# Autodesk Inventor assembly: CL7-GB-100
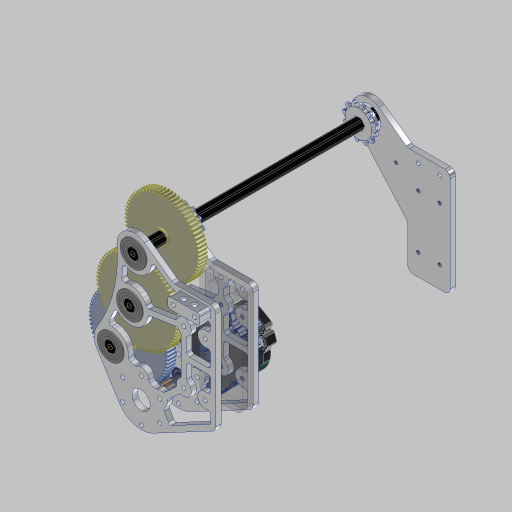
[picture p0: Inventor's stored thumbnail of the model, 512x512]
Saved by Autodesk Inventor 2023.5 (Build 275446000, 446)
## iProperties
Created: 2025-03-18
Part Number: CL7-GB-100
Document SubType Name: Assembly
Designer: slick
Mass: 1483.84 g
Surface Area: 2349.97 cm^2
Volume: 652.786 cm^3
Density: 2.27309 g/cm^3
Author: slick
## Documents named in this file (17)
- C:\Users\slick\OneDrive\Desktop\2025-ReefScape---CAD\Climber\CL7\CL-GB\CL7-GB-100.iam
- C:\Users\slick\OneDrive\Desktop\2025-ReefScape---CAD\Climber\CL7\CL-GB\CL7-GB-001.ipt
- C:\Users\slick\OneDrive\Desktop\2025-ReefScape---CAD\Climber\CL7\CL-GB\CL7-GB-002.ipt
- C:\Users\slick\OneDrive\Desktop\2025-ReefScape---CAD\Climber\CL7\CL-GB\CL7-GB-003.ipt
- C:\Users\slick\OneDrive\Desktop\2025-ReefScape---CAD\COMMON PARTS\MOTORS\Kracken with Cover and Boards.iam
- C:\Users\slick\OneDrive\Desktop\2025-ReefScape---CAD\COMMON PARTS\BEARINGS\13_75mm_1_2_ThunderHex_ID_x_1_125_OD_x_0_313_WD_Flanged_Bearing_217-4006_MIR.ipt
- C:\Users\slick\OneDrive\Desktop\2025-ReefScape---CAD\COMMON PARTS\GEARS\20dp .5 hex\72t_Aluminum_Spur_Gear_20_DP_1_2_Hex_Bore_217-3576.ipt
- C:\Users\slick\OneDrive\Desktop\2025-ReefScape---CAD\COMMON PARTS\GEARS\20dp .5 hex\18t_Aluminum_Spur_Gear_20_DP_1_2_Hex_Bore_217-3209.ipt
- C:\Users\slick\OneDrive\Desktop\2025-ReefScape---CAD\COMMON PARTS\GEARS\20dp .5 hex\74t_Aluminum_Spur_Gear_20_DP_1_2_Hex_Bore_217-5478.ipt
- C:\Users\slick\OneDrive\Desktop\2025-ReefScape---CAD\COMMON PARTS\GEARS\20dp .5 hex\20t_Aluminum_Spur_Gear_20_DP_1_2_Hex_Bore_217-2702.ipt
- C:\Users\slick\OneDrive\Desktop\2025-ReefScape---CAD\COMMON PARTS\GEARS\20dp .5 hex\68t_Aluminum_Spur_Gear_20_DP_1_2_Hex_Bore_217-5477.ipt
- C:\Users\slick\OneDrive\Desktop\2025-ReefScape---CAD\COMMON PARTS\GEARS\WCP-1006\WCP-1006.ipt
- C:\Users\slick\OneDrive\Desktop\2025-ReefScape---CAD\Climber\CL7\CL-GB\CL7-GB-004.ipt
- C:\Users\slick\OneDrive\Desktop\2025-ReefScape---CAD\COMMON PARTS\SPROCKETS\35\12t_Aluminum_Hub_Sprocket_35_Chain_1_2_Hex_Bore_217-2662.ipt
- C:\Users\slick\OneDrive\Desktop\2025-ReefScape---CAD\Climber\CL7\CL-GB\CL7-GB-006.ipt
- C:\Users\slick\OneDrive\Desktop\2025-ReefScape---CAD\Climber\CL7\CL-GB\CL7-GB-007.ipt
- C:\Users\slick\OneDrive\Desktop\2025-ReefScape---CAD\Climber\CL7\CL-GB\CL7-GB-008.ipt
## Components (24 placed, 16 different names)
1. CL7-GB-001:1 — Mate:2, Insert:6, Insert:7, Insert:8, Flush:5, Mate:18, Mate:19, Insert:14, Insert:15, Insert:16, Mate:23, Flush:12, Mate:34
2. CL7-GB-002:1 — Mate:2, Flush:1, Insert:9, Insert:10, Insert:11, Flush:5, Mate:23, Insert:17, Insert:18, Mate:33
3. CL7-GB-003:1 — Insert:1, Insert:2, Flush:1, Insert:15, Insert:16
4. CL7-GB-003:2 — Insert:1, Insert:2
5. Kracken with Cover and Boards:1 [sub-assembly] — Mate:18, Mate:19, Insert:14, Mate:20
6. 13_75mm_1_2_ThunderHex_ID_x_1_125_OD_x_0_313_WD_Flanged_Bearing_217-4006_MIR:1 — Insert:8, Mate:5, Mate:27, Flush:6
7. 13_75mm_1_2_ThunderHex_ID_x_1_125_OD_x_0_313_WD_Flanged_Bearing_217-4006_MIR:2 — Insert:7, Mate:28, Flush:7
8. 13_75mm_1_2_ThunderHex_ID_x_1_125_OD_x_0_313_WD_Flanged_Bearing_217-4006_MIR:3 — Insert:6, Mate:21, Mate:24
9. 13_75mm_1_2_ThunderHex_ID_x_1_125_OD_x_0_313_WD_Flanged_Bearing_217-4006_MIR:4 — Insert:11, Mate:12, Mate:29, Mate:30, Flush:11
10. 13_75mm_1_2_ThunderHex_ID_x_1_125_OD_x_0_313_WD_Flanged_Bearing_217-4006_MIR:5 — Insert:10, Mate:9, Mate:10, Mate:26
11. 13_75mm_1_2_ThunderHex_ID_x_1_125_OD_x_0_313_WD_Flanged_Bearing_217-4006_MIR:6 — Insert:9
12. 72t_Aluminum_Spur_Gear_20_DP_1_2_Hex_Bore_217-3576:1 — Mate:5, Mate:7, Flush:4, Mate:22
13. 18t_Aluminum_Spur_Gear_20_DP_1_2_Hex_Bore_217-3209:1 — Mate:7, Flush:2, Mate:22
14. 74t_Aluminum_Spur_Gear_20_DP_1_2_Hex_Bore_217-5478:1 — Mate:9, Flush:2, Mate:26
15. 20t_Aluminum_Spur_Gear_20_DP_1_2_Hex_Bore_217-2702:1 — Mate:10, Flush:3
16. 68t_Aluminum_Spur_Gear_20_DP_1_2_Hex_Bore_217-5477:1 — Mate:12, Flush:3, Mate:21
17. WCP-1006:1 — Flush:4, Mate:20
18. CL7-GB-004:1 — Insert:17, Insert:18
19. 12t_Aluminum_Hub_Sprocket_35_Chain_1_2_Hex_Bore_217-2662:1 — Mate:24, Mate:29
20. CL7-GB-006:1 — Mate:27, Flush:6
21. CL7-GB-006:2 — Mate:28, Flush:7
22. CL7-GB-007:1 — Mate:30, Flush:11, Mate:32
23. 12t_Aluminum_Hub_Sprocket_35_Chain_1_2_Hex_Bore_217-2662:2 — Mate:32
24. CL7-GB-008:1 — Mate:33, Flush:12, Mate:34
## Relationships (43: Mate 21, Insert 13, Flush 9)
- Insert:1: CL7-GB-003:1 ↔ CL7-GB-003:2
- Insert:2: CL7-GB-003:1 ↔ CL7-GB-003:2
- Mate:2: CL7-GB-001:1 ↔ CL7-GB-002:1
- Flush:1: CL7-GB-002:1 ↔ CL7-GB-003:1
- Insert:6: CL7-GB-001:1 ↔ 13_75mm_1_2_ThunderHex_ID_x_1_125_OD_x_0_313_WD_Flanged_Bearing_217-4006_MIR:3
- Insert:7: CL7-GB-001:1 ↔ 13_75mm_1_2_ThunderHex_ID_x_1_125_OD_x_0_313_WD_Flanged_Bearing_217-4006_MIR:2
- Insert:8: CL7-GB-001:1 ↔ 13_75mm_1_2_ThunderHex_ID_x_1_125_OD_x_0_313_WD_Flanged_Bearing_217-4006_MIR:1
- Insert:9: CL7-GB-002:1 ↔ 13_75mm_1_2_ThunderHex_ID_x_1_125_OD_x_0_313_WD_Flanged_Bearing_217-4006_MIR:6
- Insert:10: CL7-GB-002:1 ↔ 13_75mm_1_2_ThunderHex_ID_x_1_125_OD_x_0_313_WD_Flanged_Bearing_217-4006_MIR:5
- Insert:11: CL7-GB-002:1 ↔ 13_75mm_1_2_ThunderHex_ID_x_1_125_OD_x_0_313_WD_Flanged_Bearing_217-4006_MIR:4
- Mate:5: 13_75mm_1_2_ThunderHex_ID_x_1_125_OD_x_0_313_WD_Flanged_Bearing_217-4006_MIR:1 ↔ 72t_Aluminum_Spur_Gear_20_DP_1_2_Hex_Bore_217-3576:1
- Mate:7: 72t_Aluminum_Spur_Gear_20_DP_1_2_Hex_Bore_217-3576:1 ↔ 18t_Aluminum_Spur_Gear_20_DP_1_2_Hex_Bore_217-3209:1
- Mate:9: 13_75mm_1_2_ThunderHex_ID_x_1_125_OD_x_0_313_WD_Flanged_Bearing_217-4006_MIR:5 ↔ 74t_Aluminum_Spur_Gear_20_DP_1_2_Hex_Bore_217-5478:1
- Flush:2: 18t_Aluminum_Spur_Gear_20_DP_1_2_Hex_Bore_217-3209:1 ↔ 74t_Aluminum_Spur_Gear_20_DP_1_2_Hex_Bore_217-5478:1
- Mate:10: 13_75mm_1_2_ThunderHex_ID_x_1_125_OD_x_0_313_WD_Flanged_Bearing_217-4006_MIR:5 ↔ 20t_Aluminum_Spur_Gear_20_DP_1_2_Hex_Bore_217-2702:1
- Mate:12: 13_75mm_1_2_ThunderHex_ID_x_1_125_OD_x_0_313_WD_Flanged_Bearing_217-4006_MIR:4 ↔ 68t_Aluminum_Spur_Gear_20_DP_1_2_Hex_Bore_217-5477:1
- Flush:3: 20t_Aluminum_Spur_Gear_20_DP_1_2_Hex_Bore_217-2702:1 ↔ 68t_Aluminum_Spur_Gear_20_DP_1_2_Hex_Bore_217-5477:1
- Flush:4 (6.35 mm): 72t_Aluminum_Spur_Gear_20_DP_1_2_Hex_Bore_217-3576:1 ↔ WCP-1006:1
- Flush:5: CL7-GB-001:1 ↔ CL7-GB-002:1
- Mate:18: CL7-GB-001:1 ↔ Kracken with Cover and Boards:1
- Mate:19: CL7-GB-001:1 ↔ Kracken with Cover and Boards:1
- Insert:14: CL7-GB-001:1 ↔ Kracken with Cover and Boards:1
- Mate:20: Kracken with Cover and Boards:1 ↔ WCP-1006:1
- Mate:21: 13_75mm_1_2_ThunderHex_ID_x_1_125_OD_x_0_313_WD_Flanged_Bearing_217-4006_MIR:3 ↔ 68t_Aluminum_Spur_Gear_20_DP_1_2_Hex_Bore_217-5477:1
- Mate:22: 72t_Aluminum_Spur_Gear_20_DP_1_2_Hex_Bore_217-3576:1 ↔ 18t_Aluminum_Spur_Gear_20_DP_1_2_Hex_Bore_217-3209:1
- Insert:15: CL7-GB-001:1 ↔ CL7-GB-003:1
- Insert:16: CL7-GB-001:1 ↔ CL7-GB-003:1
- Mate:23 (38.1 mm): CL7-GB-001:1 ↔ CL7-GB-002:1
- Insert:17: CL7-GB-002:1 ↔ CL7-GB-004:1
- Insert:18: CL7-GB-002:1 ↔ CL7-GB-004:1
- Mate:24: 13_75mm_1_2_ThunderHex_ID_x_1_125_OD_x_0_313_WD_Flanged_Bearing_217-4006_MIR:3 ↔ 12t_Aluminum_Hub_Sprocket_35_Chain_1_2_Hex_Bore_217-2662:1
- Mate:26: 13_75mm_1_2_ThunderHex_ID_x_1_125_OD_x_0_313_WD_Flanged_Bearing_217-4006_MIR:5 ↔ 74t_Aluminum_Spur_Gear_20_DP_1_2_Hex_Bore_217-5478:1
- Mate:27: 13_75mm_1_2_ThunderHex_ID_x_1_125_OD_x_0_313_WD_Flanged_Bearing_217-4006_MIR:1 ↔ CL7-GB-006:1
- Flush:6: 13_75mm_1_2_ThunderHex_ID_x_1_125_OD_x_0_313_WD_Flanged_Bearing_217-4006_MIR:1 ↔ CL7-GB-006:1
- Mate:28: 13_75mm_1_2_ThunderHex_ID_x_1_125_OD_x_0_313_WD_Flanged_Bearing_217-4006_MIR:2 ↔ CL7-GB-006:2
- Flush:7: 13_75mm_1_2_ThunderHex_ID_x_1_125_OD_x_0_313_WD_Flanged_Bearing_217-4006_MIR:2 ↔ CL7-GB-006:2
- Mate:29 (-66.675 mm): 13_75mm_1_2_ThunderHex_ID_x_1_125_OD_x_0_313_WD_Flanged_Bearing_217-4006_MIR:4 ↔ 12t_Aluminum_Hub_Sprocket_35_Chain_1_2_Hex_Bore_217-2662:1
- Mate:30: 13_75mm_1_2_ThunderHex_ID_x_1_125_OD_x_0_313_WD_Flanged_Bearing_217-4006_MIR:4 ↔ CL7-GB-007:1
- Flush:11: 13_75mm_1_2_ThunderHex_ID_x_1_125_OD_x_0_313_WD_Flanged_Bearing_217-4006_MIR:4 ↔ CL7-GB-007:1
- Mate:32: CL7-GB-007:1 ↔ 12t_Aluminum_Hub_Sprocket_35_Chain_1_2_Hex_Bore_217-2662:2
- Mate:33: CL7-GB-002:1 ↔ CL7-GB-008:1
- Flush:12: CL7-GB-001:1 ↔ CL7-GB-008:1
- Mate:34 (228.6 mm): CL7-GB-001:1 ↔ CL7-GB-008:1
